# Autodesk Inventor assembly: Zesilovac
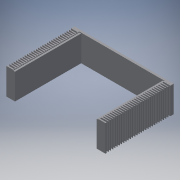
[picture p0: Inventor's stored thumbnail of the model, 180x180]
Saved by Autodesk Inventor 2019 (Build 230136000, 136)
## iProperties
Created: 2021-01-08
Part Number: Zesilovac
Material: Všeobecné
Document SubType Name: Assembly
Designer: Pokor
Author: Pokor
## Documents named in this file (3)
- D:\Disk Google\#PROJEKTY-COPY\Zesilovace\Hifi_LeachAmp\LeachAmp_3D_model\Zesilovac.iam
- D:\Disk Google\#PROJEKTY-COPY\Zesilovace\Hifi_LeachAmp\LeachAmp_3D_model\chladic.ipt
- D:\Disk Google\#PROJEKTY-COPY\Zesilovace\Hifi_LeachAmp\LeachAmp_3D_model\Predni_strana.ipt
## Components (3 placed, 2 different names)
1. chladic:1 — Proti sobě:1, Stejný směr:1, Stejný směr:2, Stejný směr:3
2. chladic:2 — Stejný směr:3, Stejný směr:4, Stejný směr:5
3. Predni_strana:1 — Proti sobě:1, Stejný směr:1, Stejný směr:2, Stejný směr:4, Stejný směr:5
## Relationships (6: Flush 5, Mate 1)
- Proti sobě:1 [Mate]: chladic:1 ↔ Predni_strana:1
- Stejný směr:1 [Flush]: chladic:1 ↔ Predni_strana:1
- Stejný směr:2 [Flush]: chladic:1 ↔ Predni_strana:1
- Stejný směr:3 [Flush]: chladic:1 ↔ chladic:2
- Stejný směr:4 [Flush]: chladic:2 ↔ Predni_strana:1
- Stejný směr:5 [Flush]: chladic:2 ↔ Predni_strana:1
